# Autodesk Inventor assembly: stand
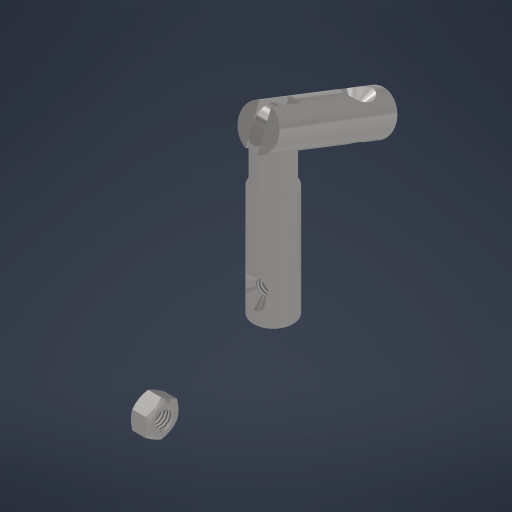
[picture p0: Inventor's stored thumbnail of the model, 512x512]
Saved by Autodesk Inventor 2023 (Build 270158000, 158)
## iProperties
Created: 2022-04-24
Part Number: stand
Document SubType Name: Assembly
Designer: Norbert Ligas
bar_lenght: 185,000 mm
pipe_lenght: 200,000 mm
Author: Norbert Ligas
## Documents named in this file (5)
- C:\Users\norbe\Repozytoria\NormalMapScanner\stand_construction\stand.iam
- C:\Users\norbe\Repozytoria\NormalMapScanner\stand_construction\parts\barrel_hinge.iam
- C:\Users\norbe\OneDrive\Dokumenty\Inventor\Content Center Files\R2023\en-US\ISO 4032(2)\ISO 4032 - M5 - ISO.ipt
- C:\Users\norbe\Repozytoria\NormalMapScanner\stand_construction\parts\bar.ipt
- C:\Users\norbe\Repozytoria\NormalMapScanner\stand_construction\parts\pipe.ipt
## Components (2 placed, 2 different names)
1. barrel_hinge:1 [sub-assembly] — Mate:2, Mate:3, Angle:1
2. ISO 4032 M5:1
## Relationships (3: Mate 2, Angle 1)
- Mate:2: barrel_hinge:1
- Mate:3: barrel_hinge:1
- Angle:1 (0 deg): barrel_hinge:1
